# Autodesk Inventor assembly: Arm Assembly 1
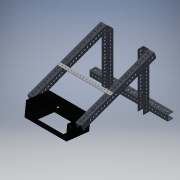
[picture p0: Inventor's stored thumbnail of the model, 180x180]
Saved by Autodesk Inventor 2016 (Build 200138000, 138)
## iProperties
Created: 2015-09-15
Part Number: Arm Assembly 1
Document SubType Name: Assembly
Designer: tbloo
Author: tbloo
## Documents named in this file (5)
- C:\Users\tbloo\Documents\GitHub\phi_robotics\3d-models\FTC_Tetrix_KOP_Block_Party\Tim Bloot Designs\Arm Assembly 1.iam
- C:\Users\tbloo\Documents\GitHub\phi_robotics\3d-models\FTC_Tetrix_KOP_Block_Party\Tetrix_Kit_FTC\Autodesk Inventor Files\tetrix_c_channel-5.ipt
- C:\Users\tbloo\Documents\GitHub\phi_robotics\3d-models\FTC_Tetrix_KOP_Block_Party\Tetrix_Kit_FTC\Autodesk Inventor Files\tetrix_c_channel-4.ipt
- C:\Users\tbloo\Documents\GitHub\phi_robotics\3d-models\FTC_Tetrix_KOP_Block_Party\Tetrix_Kit_FTC\Autodesk Inventor Files\tetrix_flat_bar-288 MM.ipt
- C:\Users\tbloo\Documents\GitHub\phi_robotics\3d-models\FTC_Tetrix_KOP_Block_Party\Tim Bloot Designs\Bucket des 1.ipt
## Components (7 placed, 4 different names)
1. tetrix_c_channel-5:1 — Rigid:1, Rigid:2
2. tetrix_c_channel-4:1 — Rigid:2, Rotational:1
3. tetrix_c_channel-4:2 — Rigid:1, Rotational:2
4. tetrix_c_channel-5:2 — Rotational:1, Rigid:4, Rotational:3
5. tetrix_c_channel-5:3 — Rotational:2, Rigid:3, Rotational:4
6. tetrix_flat_bar-288 MM:1 — Rigid:4, Rigid:3
7. Bucket des 1:1 — Rotational:3, Rotational:4
## Relationships (8: WeldJoint 4, RevoluteJoint 4)
- Rigid:1 [WeldJoint]: tetrix_c_channel-5:1 ↔ tetrix_c_channel-4:2
- Rigid:2 [WeldJoint]: tetrix_c_channel-5:1 ↔ tetrix_c_channel-4:1
- Rotational:1 [RevoluteJoint]: tetrix_c_channel-4:1 ↔ tetrix_c_channel-5:2
- Rotational:2 [RevoluteJoint]: tetrix_c_channel-4:2 ↔ tetrix_c_channel-5:3
- Rigid:4 [WeldJoint]: tetrix_c_channel-5:2 ↔ tetrix_flat_bar-288 MM:1
- Rigid:3 [WeldJoint]: tetrix_c_channel-5:3 ↔ tetrix_flat_bar-288 MM:1
- Rotational:3 [RevoluteJoint]: tetrix_c_channel-5:2 ↔ Bucket des 1:1
- Rotational:4 [RevoluteJoint]: tetrix_c_channel-5:3 ↔ Bucket des 1:1
